# Autodesk Inventor assembly: Euph Cart
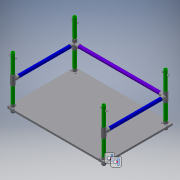
[picture p0: Inventor's stored thumbnail of the model, 180x180]
Saved by Autodesk Inventor 2018.2 (Build 222227000, 227)
## iProperties
Created: 2018-02-07
Part Number: Euph Cart
Document SubType Name: Assembly
Designer: owner
Author: owner
## Documents named in this file (10)
- Z:\The Pickle\Final Carts\Euph Cart\Euph Cart.iam
- Z:\The Pickle\Final Carts\Euph Cart\Plywood Base.ipt
- Z:\The Pickle\Inventor Pipe Parts\Formufit Fittings\4-way Tee 1 Inch.ipt
- Z:\The Pickle\Inventor Pipe Parts\Formufit Fittings\Tee 1 Inch.ipt
- Z:\The Pickle\Inventor Pipe Parts\Formufit Fittings\Wood Mount 1 Inch.ipt
- Z:\The Pickle\Final Carts\Euph Cart\Pipe 1.ipt
- Z:\The Pickle\Final Carts\Euph Cart\Pipe 2.ipt
- Z:\The Pickle\Final Carts\Euph Cart\Pipe 3.ipt
- Z:\The Pickle\Final Carts\Locking Mech\Eyebolt.ipt
- Z:\The Pickle\Final Carts\Locking Mech\Eyebolt Nut.ipt
## Components (32 placed, 9 different names)
1. 4-way Tee 1 Inch:2 — Insert:37, Insert:38, Insert:39, Insert:40, Mate:4
2. Tee 1 Inch:3 — Insert:43, Insert:44, Insert:46, Mate:5
3. Tee 1 Inch:4 — Insert:41, Insert:42, Insert:45
4. Pipe 1:2 — Insert:39, Insert:43
5. Plywood Base:2 — Tangent:4, Tangent:5, Mate:7, Mate:8, Tangent:6, Tangent:7, Tangent:8, Mate:9, Tangent:9, Tangent:10, Tangent:11, Mate:10, Tangent:12, Tangent:13, Mate:11, Tangent:14, Tangent:15
6. 4-way Tee 1 Inch:5
7. Wood Mount 1 Inch:9
8. Wood Mount 1 Inch:10
9. Wood Mount 1 Inch:11 — Tangent:4, Mate:6, Tangent:5, Mate:7
10. Wood Mount 1 Inch:12
11. Pipe 1:3 — Insert:42
12. Pipe 2:4 — Insert:38
13. Pipe 3:9 — Insert:37
14. Pipe 3:10
15. Pipe 3:11 — Insert:41
16. Pipe 3:12 — Cylindrical:4
17. Pipe 3:13 — Insert:40, Cylindrical:1
18. Pipe 3:14 — Insert:46, Cylindrical:2
19. Pipe 3:15 — Insert:45, Cylindrical:3
20. Pipe 3:16 — Insert:44
21. Eyebolt:1 — Cylindrical:1, Insert:47
22. Eyebolt:2 — Cylindrical:3, Insert:48
23. Eyebolt:3 — Cylindrical:4, Cylindrical:7
24. Eyebolt:4 — Cylindrical:2, Cylindrical:5
25. Eyebolt Nut:1 — Cylindrical:7
26. Eyebolt Nut:2 — Insert:47
27. Eyebolt Nut:3 — Insert:48
28. Eyebolt Nut:4 — Cylindrical:5
29. Wood Mount 1 Inch:13 — Mate:6, Mate:8, Tangent:6, Tangent:7, Tangent:8
30. Wood Mount 1 Inch:15 — Mate:10, Tangent:12, Tangent:13
31. Wood Mount 1 Inch:16 — Mate:11, Tangent:14, Tangent:15
32. Wood Mount 1 Inch:17 — Mate:9, Tangent:9, Tangent:10, Tangent:11
## Relationships (46: Insert 19, Tangent 13, Mate 8, CylindricalJoint 6)
- [Tangent]: Plywood Base:2 ↔ Wood Mount 1 Inch:11
- [Insert]: 4-way Tee 1 Inch:5 ↔ Pipe 1:3
- [Insert]: 4-way Tee 1 Inch:5 ↔ Pipe 2:4
- [Insert]: 4-way Tee 1 Inch:5 ↔ Pipe 3:10
- [Insert]: Wood Mount 1 Inch:12 ↔ Pipe 3:9
- [Insert]: Wood Mount 1 Inch:10 ↔ Pipe 3:10
- [Insert]: Wood Mount 1 Inch:9 ↔ Pipe 3:11
- [Insert]: 4-way Tee 1 Inch:5 ↔ Pipe 3:12
- Insert:37: 4-way Tee 1 Inch:2 ↔ Pipe 3:9
- Insert:38: 4-way Tee 1 Inch:2 ↔ Pipe 2:4
- Insert:39: 4-way Tee 1 Inch:2 ↔ Pipe 1:2
- Insert:40: 4-way Tee 1 Inch:2 ↔ Pipe 3:13
- Insert:41: Tee 1 Inch:4 ↔ Pipe 3:11
- Insert:42: Tee 1 Inch:4 ↔ Pipe 1:3
- Insert:43: Tee 1 Inch:3 ↔ Pipe 1:2
- Insert:44: Tee 1 Inch:3 ↔ Pipe 3:16
- Insert:45: Tee 1 Inch:4 ↔ Pipe 3:15
- Insert:46: Tee 1 Inch:3 ↔ Pipe 3:14
- Mate:4: 4-way Tee 1 Inch:2
- Mate:5: Tee 1 Inch:3
- Cylindrical:1: Pipe 3:13 ↔ Eyebolt:1
- Cylindrical:2: Pipe 3:14 ↔ Eyebolt:4
- Cylindrical:3: Pipe 3:15 ↔ Eyebolt:2
- Cylindrical:4: Pipe 3:12 ↔ Eyebolt:3
- Cylindrical:5: Eyebolt:4 ↔ Eyebolt Nut:4
- Cylindrical:7: Eyebolt:3 ↔ Eyebolt Nut:1
- Insert:47: Eyebolt:1 ↔ Eyebolt Nut:2
- Insert:48: Eyebolt:2 ↔ Eyebolt Nut:3
- Tangent:4: Plywood Base:2 ↔ Wood Mount 1 Inch:11
- Mate:6: Wood Mount 1 Inch:11 ↔ Wood Mount 1 Inch:13
- Tangent:5: Plywood Base:2 ↔ Wood Mount 1 Inch:11
- Mate:7: Plywood Base:2 ↔ Wood Mount 1 Inch:11
- Mate:8: Plywood Base:2 ↔ Wood Mount 1 Inch:13
- Tangent:6: Plywood Base:2 ↔ Wood Mount 1 Inch:13
- Tangent:7: Plywood Base:2 ↔ Wood Mount 1 Inch:13
- Tangent:8: Plywood Base:2 ↔ Wood Mount 1 Inch:13
- Mate:9: Plywood Base:2 ↔ Wood Mount 1 Inch:17
- Tangent:9: Plywood Base:2 ↔ Wood Mount 1 Inch:17
- Tangent:10: Plywood Base:2 ↔ Wood Mount 1 Inch:17
- Tangent:11: Plywood Base:2 ↔ Wood Mount 1 Inch:17
- Mate:10: Plywood Base:2 ↔ Wood Mount 1 Inch:15
- Tangent:12: Plywood Base:2 ↔ Wood Mount 1 Inch:15
- Tangent:13: Plywood Base:2 ↔ Wood Mount 1 Inch:15
- Mate:11: Plywood Base:2 ↔ Wood Mount 1 Inch:16
- Tangent:14: Plywood Base:2 ↔ Wood Mount 1 Inch:16
- Tangent:15: Plywood Base:2 ↔ Wood Mount 1 Inch:16
## Named parameters: d21_d12 = 0 mm, d23_d14 = 0 mm, d24_d15 = 0 mm, d25_d16 = 0 mm, d28_d19 = 0 mm, d30_d1 = 0 mm, d37_d8 = 0 mm, d38_d9 = 0 mm
